# Autodesk Inventor assembly: Catapult Launcher
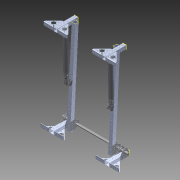
[picture p0: Inventor's stored thumbnail of the model, 180x180]
Saved by Autodesk Inventor 2014 (Build 180170000, 170)
## iProperties
Created: 2014-01-17
Part Number: Catapult Launcher
Document SubType Name: Assembly
Designer: Andrew Toennies
Mass: 1552.27 g
Surface Area: 5150.08 cm^2
Volume: 383.1 cm^3
Density: 4.05187 g/cm^3
Author: Andrew Toennies
## Documents named in this file (10)
- C:\Users\Andrew Toennies\Documents\GitHub\2014buildCAD\New Shooter\Catapult Launcher.iam
- C:\Users\Andrew Toennies\Documents\GitHub\2014buildCAD\New Shooter\Vex Pro 1x1 rectangular tubing 7 in length.ipt
- C:\Users\Andrew Toennies\Documents\GitHub\2014buildCAD\New Shooter\Vex Pro Side Bearing Gusset.ipt
- C:\Users\Andrew Toennies\Documents\GitHub\2014buildCAD\New Shooter\Vex Pro Corner Gusset.ipt
- C:\Users\Andrew Toennies\Documents\GitHub\2014buildCAD\New Shooter\Bearing ID 0.500 Hex OD 1.125.ipt
- C:\Users\Andrew Toennies\Documents\GitHub\2014buildCAD\New Shooter\Shaft (Steel 0.500 Hex).ipt
- C:\Users\Andrew Toennies\Documents\GitHub\2014buildCAD\New Shooter\Vex Pro 1x1 rectangular tubing 27 in length.ipt
- C:\Users\Andrew Toennies\Documents\GitHub\2014buildCAD\New Shooter\098-DP(D-167)(F,D-166-1).iam
- C:\Users\Andrew Toennies\Documents\GitHub\2014buildCAD\New Shooter\D-168.ipt
- C:\Users\Andrew Toennies\Documents\GitHub\2014buildCAD\New Shooter\D-9966.ipt
## Components (35 placed, 9 different names)
1. Shaft (Steel 0.500 Hex):1 — Mate:34, Mate:35, Flush:12
2. Vex Pro Corner Gusset:5 — Mate:88, Mate:89, Mate:90, Flush:13, Flush:14
3. Vex Pro Corner Gusset:6 — Mate:85, Mate:86, Mate:87
4. Vex Pro Corner Gusset:7 — Mate:91, Mate:92, Mate:93
5. Vex Pro Corner Gusset:8 — Mate:94, Mate:95, Mate:96
6. D-168:1 — Mate:100, Mate:101, Mate:102
7. D-9966:1 — Mate:103, Mate:104, Mate:105
8. Vex Pro 1x1 rectangular tubing 7 in length:1 — Flush:1, Flush:2, Mate:1, Mate:8, Mate:9, Mate:10, Mate:11, Mate:12, Mate:13, Mate:20, Mate:21, Mate:22, Mate:23, Mate:24, Mate:25, Mate:37
9. Vex Pro 1x1 rectangular tubing 7 in length:2 — Flush:1, Flush:2, Mate:1, Mate:2, Mate:3, Mate:4, Mate:5, Mate:6, Mate:7, Mate:14, Mate:15, Mate:16, Mate:17, Mate:18, Mate:19, Flush:6, Mate:36, Flush:7
10. Vex Pro Side Bearing Gusset:1 — Mate:2, Mate:3, Mate:4, Mate:26, Mate:27
11. Vex Pro Side Bearing Gusset:2 — Mate:5, Mate:6, Mate:7, Mate:28, Mate:29
12. Vex Pro Side Bearing Gusset:3 — Mate:11, Mate:12, Mate:13, Mate:32, Mate:33
13. Vex Pro Side Bearing Gusset:4 — Mate:8, Mate:9, Mate:10, Mate:30, Mate:31
14. Vex Pro Corner Gusset:1 — Mate:17, Mate:18, Mate:19
15. Vex Pro Corner Gusset:2 — Mate:14, Mate:15, Mate:16
16. Vex Pro Corner Gusset:3 — Mate:20, Mate:21, Mate:22
17. Vex Pro Corner Gusset:4 — Mate:23, Mate:24, Mate:25
18. Bearing ID 0.500 Hex OD 1.125:1 — Mate:28, Mate:29, Flush:3, Flush:5
19. Bearing ID 0.500 Hex OD 1.125:2 — Mate:26, Mate:27, Flush:3, Mate:34, Mate:35, Mate:44
20. Bearing ID 0.500 Hex OD 1.125:3 — Mate:30, Mate:31, Flush:4, Flush:12
21. Bearing ID 0.500 Hex OD 1.125:4 — Mate:32, Mate:33, Flush:4, Flush:5, Mate:69
22. Vex Pro 1x1 rectangular tubing 7 in length:3 — Flush:6, Mate:36, Flush:7, Flush:8, Flush:9, Mate:91, Mate:92, Mate:93, Mate:94, Mate:95, Mate:96, Mate:98, Flush:16
23. Vex Pro 1x1 rectangular tubing 7 in length:5 — Flush:8, Flush:9, Mate:37, Mate:84, Mate:85, Mate:86, Mate:87, Mate:88, Mate:89, Mate:90, Mate:97
24. Vex Pro Side Bearing Gusset:5 — Mate:57, Mate:58, Mate:77, Mate:78, Mate:79
25. Vex Pro Side Bearing Gusset:6 — Mate:55, Mate:56, Mate:70, Mate:74, Mate:75
26. Vex Pro Side Bearing Gusset:7 — Mate:51, Mate:52, Mate:71, Mate:72, Mate:73
27. Vex Pro Side Bearing Gusset:8 — Mate:44, Mate:53, Mate:54, Mate:76, Mate:81, Mate:82
28. Vex Pro 1x1 rectangular tubing 27 in length:1 — Flush:10, Mate:70, Mate:71, Mate:72, Mate:73, Mate:74, Mate:75, Mate:83, Mate:84, Mate:101, Mate:102
29. Vex Pro 1x1 rectangular tubing 27 in length:2 — Flush:10, Mate:76, Mate:77, Mate:78, Mate:79, Mate:81, Mate:82, Mate:83, Mate:103, Mate:105
30. Bearing ID 0.500 Hex OD 1.125:5 — Mate:57, Mate:58, Mate:80
31. Bearing ID 0.500 Hex OD 1.125:6 — Mate:53, Mate:54, Mate:80
32. Bearing ID 0.500 Hex OD 1.125:7 — Mate:51, Mate:52, Mate:68, Mate:69
33. Bearing ID 0.500 Hex OD 1.125:8 — Mate:55, Mate:56, Mate:68
34. 098-DP(D-167)(F,D-166-1):1 [sub-assembly] — Mate:97, Flush:13, Flush:14, Flush:15, Mate:99, Mate:100
35. 098-DP(D-167)(F,D-166-1):2 [sub-assembly] — Mate:98, Flush:15, Flush:16, Mate:99, Mate:104
## Relationships (99: Mate 84, Flush 15)
- Flush:1: Vex Pro 1x1 rectangular tubing 7 in length:1 ↔ Vex Pro 1x1 rectangular tubing 7 in length:2
- Flush:2: Vex Pro 1x1 rectangular tubing 7 in length:1 ↔ Vex Pro 1x1 rectangular tubing 7 in length:2
- Mate:1 (381 mm): Vex Pro 1x1 rectangular tubing 7 in length:1 ↔ Vex Pro 1x1 rectangular tubing 7 in length:2
- Mate:2: Vex Pro 1x1 rectangular tubing 7 in length:2 ↔ Vex Pro Side Bearing Gusset:1
- Mate:3: Vex Pro 1x1 rectangular tubing 7 in length:2 ↔ Vex Pro Side Bearing Gusset:1
- Mate:4: Vex Pro 1x1 rectangular tubing 7 in length:2 ↔ Vex Pro Side Bearing Gusset:1
- Mate:5: Vex Pro 1x1 rectangular tubing 7 in length:2 ↔ Vex Pro Side Bearing Gusset:2
- Mate:6: Vex Pro 1x1 rectangular tubing 7 in length:2 ↔ Vex Pro Side Bearing Gusset:2
- Mate:7: Vex Pro 1x1 rectangular tubing 7 in length:2 ↔ Vex Pro Side Bearing Gusset:2
- Mate:8: Vex Pro 1x1 rectangular tubing 7 in length:1 ↔ Vex Pro Side Bearing Gusset:4
- Mate:9: Vex Pro 1x1 rectangular tubing 7 in length:1 ↔ Vex Pro Side Bearing Gusset:4
- Mate:10: Vex Pro 1x1 rectangular tubing 7 in length:1 ↔ Vex Pro Side Bearing Gusset:4
- Mate:11: Vex Pro 1x1 rectangular tubing 7 in length:1 ↔ Vex Pro Side Bearing Gusset:3
- Mate:12: Vex Pro 1x1 rectangular tubing 7 in length:1 ↔ Vex Pro Side Bearing Gusset:3
- Mate:13: Vex Pro 1x1 rectangular tubing 7 in length:1 ↔ Vex Pro Side Bearing Gusset:3
- Mate:14: Vex Pro 1x1 rectangular tubing 7 in length:2 ↔ Vex Pro Corner Gusset:2
- Mate:15: Vex Pro 1x1 rectangular tubing 7 in length:2 ↔ Vex Pro Corner Gusset:2
- Mate:16: Vex Pro 1x1 rectangular tubing 7 in length:2 ↔ Vex Pro Corner Gusset:2
- Mate:17: Vex Pro 1x1 rectangular tubing 7 in length:2 ↔ Vex Pro Corner Gusset:1
- Mate:18: Vex Pro 1x1 rectangular tubing 7 in length:2 ↔ Vex Pro Corner Gusset:1
- Mate:19: Vex Pro 1x1 rectangular tubing 7 in length:2 ↔ Vex Pro Corner Gusset:1
- Mate:20: Vex Pro 1x1 rectangular tubing 7 in length:1 ↔ Vex Pro Corner Gusset:3
- Mate:21: Vex Pro 1x1 rectangular tubing 7 in length:1 ↔ Vex Pro Corner Gusset:3
- Mate:22: Vex Pro 1x1 rectangular tubing 7 in length:1 ↔ Vex Pro Corner Gusset:3
- Mate:23: Vex Pro 1x1 rectangular tubing 7 in length:1 ↔ Vex Pro Corner Gusset:4
- Mate:24: Vex Pro 1x1 rectangular tubing 7 in length:1 ↔ Vex Pro Corner Gusset:4
- Mate:25: Vex Pro 1x1 rectangular tubing 7 in length:1 ↔ Vex Pro Corner Gusset:4
- Mate:26: Vex Pro Side Bearing Gusset:1 ↔ Bearing ID 0.500 Hex OD 1.125:2
- Mate:27: Vex Pro Side Bearing Gusset:1 ↔ Bearing ID 0.500 Hex OD 1.125:2
- Mate:28: Vex Pro Side Bearing Gusset:2 ↔ Bearing ID 0.500 Hex OD 1.125:1
- Mate:29: Vex Pro Side Bearing Gusset:2 ↔ Bearing ID 0.500 Hex OD 1.125:1
- Flush:3: Bearing ID 0.500 Hex OD 1.125:1 ↔ Bearing ID 0.500 Hex OD 1.125:2
- Mate:30: Vex Pro Side Bearing Gusset:4 ↔ Bearing ID 0.500 Hex OD 1.125:3
- Mate:31: Vex Pro Side Bearing Gusset:4 ↔ Bearing ID 0.500 Hex OD 1.125:3
- Mate:32: Vex Pro Side Bearing Gusset:3 ↔ Bearing ID 0.500 Hex OD 1.125:4
- Mate:33: Vex Pro Side Bearing Gusset:3 ↔ Bearing ID 0.500 Hex OD 1.125:4
- Flush:4: Bearing ID 0.500 Hex OD 1.125:3 ↔ Bearing ID 0.500 Hex OD 1.125:4
- Flush:5: Bearing ID 0.500 Hex OD 1.125:1 ↔ Bearing ID 0.500 Hex OD 1.125:4
- Mate:34: Shaft (Steel 0.500 Hex):1 ↔ Bearing ID 0.500 Hex OD 1.125:2
- Mate:35: Shaft (Steel 0.500 Hex):1 ↔ Bearing ID 0.500 Hex OD 1.125:2
- Flush:6: Vex Pro 1x1 rectangular tubing 7 in length:2 ↔ Vex Pro 1x1 rectangular tubing 7 in length:3
- Mate:36: Vex Pro 1x1 rectangular tubing 7 in length:2 ↔ Vex Pro 1x1 rectangular tubing 7 in length:3
- Flush:7 (-660.4 mm): Vex Pro 1x1 rectangular tubing 7 in length:2 ↔ Vex Pro 1x1 rectangular tubing 7 in length:3
- Flush:8: Vex Pro 1x1 rectangular tubing 7 in length:3 ↔ Vex Pro 1x1 rectangular tubing 7 in length:5
- Flush:9: Vex Pro 1x1 rectangular tubing 7 in length:3 ↔ Vex Pro 1x1 rectangular tubing 7 in length:5
- Mate:37: Vex Pro 1x1 rectangular tubing 7 in length:1 ↔ Vex Pro 1x1 rectangular tubing 7 in length:5
- Flush:10: Vex Pro 1x1 rectangular tubing 27 in length:1 ↔ Vex Pro 1x1 rectangular tubing 27 in length:2
- Mate:44: Bearing ID 0.500 Hex OD 1.125:2 ↔ Vex Pro Side Bearing Gusset:8
- Mate:51: Vex Pro Side Bearing Gusset:7 ↔ Bearing ID 0.500 Hex OD 1.125:7
- Mate:52: Vex Pro Side Bearing Gusset:7 ↔ Bearing ID 0.500 Hex OD 1.125:7
- Mate:53: Vex Pro Side Bearing Gusset:8 ↔ Bearing ID 0.500 Hex OD 1.125:6
- Mate:54: Vex Pro Side Bearing Gusset:8 ↔ Bearing ID 0.500 Hex OD 1.125:6
- Mate:55: Vex Pro Side Bearing Gusset:6 ↔ Bearing ID 0.500 Hex OD 1.125:8
- Mate:56: Vex Pro Side Bearing Gusset:6 ↔ Bearing ID 0.500 Hex OD 1.125:8
- Mate:57: Vex Pro Side Bearing Gusset:5 ↔ Bearing ID 0.500 Hex OD 1.125:5
- Mate:58: Vex Pro Side Bearing Gusset:5 ↔ Bearing ID 0.500 Hex OD 1.125:5
- Flush:12 (-25.4 mm): Shaft (Steel 0.500 Hex):1 ↔ Bearing ID 0.500 Hex OD 1.125:3
- Mate:68: Bearing ID 0.500 Hex OD 1.125:7 ↔ Bearing ID 0.500 Hex OD 1.125:8
- Mate:69: Bearing ID 0.500 Hex OD 1.125:4 ↔ Bearing ID 0.500 Hex OD 1.125:7
- Mate:70: Vex Pro Side Bearing Gusset:6 ↔ Vex Pro 1x1 rectangular tubing 27 in length:1
- Mate:71: Vex Pro Side Bearing Gusset:7 ↔ Vex Pro 1x1 rectangular tubing 27 in length:1
- Mate:72: Vex Pro Side Bearing Gusset:7 ↔ Vex Pro 1x1 rectangular tubing 27 in length:1
- Mate:73: Vex Pro Side Bearing Gusset:7 ↔ Vex Pro 1x1 rectangular tubing 27 in length:1
- Mate:74: Vex Pro Side Bearing Gusset:6 ↔ Vex Pro 1x1 rectangular tubing 27 in length:1
- Mate:75: Vex Pro Side Bearing Gusset:6 ↔ Vex Pro 1x1 rectangular tubing 27 in length:1
- Mate:76: Vex Pro Side Bearing Gusset:8 ↔ Vex Pro 1x1 rectangular tubing 27 in length:2
- Mate:77: Vex Pro Side Bearing Gusset:5 ↔ Vex Pro 1x1 rectangular tubing 27 in length:2
- Mate:78: Vex Pro Side Bearing Gusset:5 ↔ Vex Pro 1x1 rectangular tubing 27 in length:2
- Mate:79: Vex Pro Side Bearing Gusset:5 ↔ Vex Pro 1x1 rectangular tubing 27 in length:2
- Mate:80: Bearing ID 0.500 Hex OD 1.125:5 ↔ Bearing ID 0.500 Hex OD 1.125:6
- Mate:81: Vex Pro Side Bearing Gusset:8 ↔ Vex Pro 1x1 rectangular tubing 27 in length:2
- Mate:82: Vex Pro Side Bearing Gusset:8 ↔ Vex Pro 1x1 rectangular tubing 27 in length:2
- Mate:83 (279.4 mm): Vex Pro 1x1 rectangular tubing 27 in length:1 ↔ Vex Pro 1x1 rectangular tubing 27 in length:2
- Mate:84: Vex Pro 1x1 rectangular tubing 7 in length:5 ↔ Vex Pro 1x1 rectangular tubing 27 in length:1
- Mate:85: Vex Pro Corner Gusset:6 ↔ Vex Pro 1x1 rectangular tubing 7 in length:5
- Mate:86: Vex Pro Corner Gusset:6 ↔ Vex Pro 1x1 rectangular tubing 7 in length:5
- Mate:87: Vex Pro Corner Gusset:6 ↔ Vex Pro 1x1 rectangular tubing 7 in length:5
- Mate:88: Vex Pro Corner Gusset:5 ↔ Vex Pro 1x1 rectangular tubing 7 in length:5
- Mate:89: Vex Pro Corner Gusset:5 ↔ Vex Pro 1x1 rectangular tubing 7 in length:5
- Mate:90: Vex Pro Corner Gusset:5 ↔ Vex Pro 1x1 rectangular tubing 7 in length:5
- Mate:91: Vex Pro Corner Gusset:7 ↔ Vex Pro 1x1 rectangular tubing 7 in length:3
- Mate:92: Vex Pro Corner Gusset:7 ↔ Vex Pro 1x1 rectangular tubing 7 in length:3
- Mate:93: Vex Pro Corner Gusset:7 ↔ Vex Pro 1x1 rectangular tubing 7 in length:3
- Mate:94: Vex Pro Corner Gusset:8 ↔ Vex Pro 1x1 rectangular tubing 7 in length:3
- Mate:95: Vex Pro Corner Gusset:8 ↔ Vex Pro 1x1 rectangular tubing 7 in length:3
- Mate:96: Vex Pro Corner Gusset:8 ↔ Vex Pro 1x1 rectangular tubing 7 in length:3
- Mate:97: Vex Pro 1x1 rectangular tubing 7 in length:5 ↔ 098-DP(D-167)(F,D-166-1):1
- Flush:13 (6.35 mm): Vex Pro Corner Gusset:5 ↔ 098-DP(D-167)(F,D-166-1):1
- Flush:14: Vex Pro Corner Gusset:5 ↔ 098-DP(D-167)(F,D-166-1):1
- Mate:98: Vex Pro 1x1 rectangular tubing 7 in length:3 ↔ 098-DP(D-167)(F,D-166-1):2
- Flush:15: 098-DP(D-167)(F,D-166-1):1 ↔ 098-DP(D-167)(F,D-166-1):2
- Flush:16: Vex Pro 1x1 rectangular tubing 7 in length:3 ↔ 098-DP(D-167)(F,D-166-1):2
- Mate:99: 098-DP(D-167)(F,D-166-1):1 ↔ 098-DP(D-167)(F,D-166-1):2
- Mate:100: D-168:1 ↔ 098-DP(D-167)(F,D-166-1):1
- Mate:101: D-168:1 ↔ Vex Pro 1x1 rectangular tubing 27 in length:1
- Mate:102 (3.175 mm): D-168:1 ↔ Vex Pro 1x1 rectangular tubing 27 in length:1
- Mate:103: D-9966:1 ↔ Vex Pro 1x1 rectangular tubing 27 in length:2
- Mate:104: D-9966:1 ↔ 098-DP(D-167)(F,D-166-1):2
- Mate:105 (3.175 mm): D-9966:1 ↔ Vex Pro 1x1 rectangular tubing 27 in length:2
